# Autodesk Inventor assembly: case
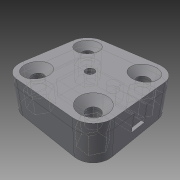
[picture p0: Inventor's stored thumbnail of the model, 180x180]
Saved by Autodesk Inventor 2014 (Build 180170000, 170)
## iProperties
Created: 2016-03-15
Part Number: case
Document SubType Name: Assembly
Designer: buben
Author: buben
## Documents named in this file (3)
- C:\Users\buben\Documents\bmp180-case\case\assemblies\case.iam
- C:\Users\buben\Documents\bmp180-case\case\parts\bottom.ipt
- C:\Users\buben\Documents\bmp180-case\case\parts\top.ipt
## Components (2 placed, 2 different names)
1. bottom:1 — Mate:1, Flush:1, Mate:2, Mate:3, Mate:4, Mate:5
2. top:1 — Mate:3, Mate:4, Mate:5
## Relationships (6: Mate 5, Flush 1)
- Mate:1: bottom:1
- Flush:1: bottom:1
- Mate:2: bottom:1
- Mate:3: bottom:1 ↔ top:1
- Mate:4: bottom:1 ↔ top:1
- Mate:5: bottom:1 ↔ top:1
